# Autodesk Inventor assembly: fourbardraft
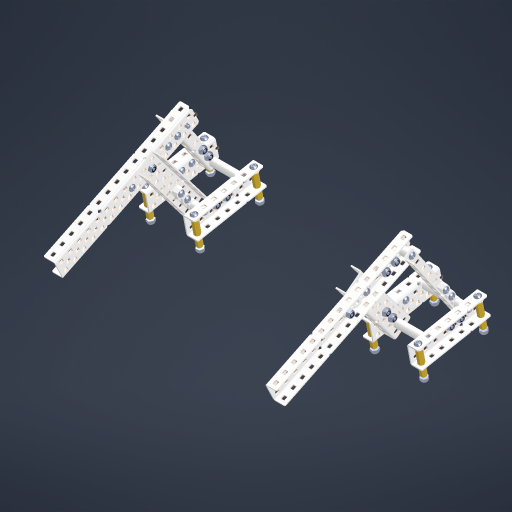
[picture p0: Inventor's stored thumbnail of the model, 512x512]
Saved by Autodesk Inventor 2023 (Build 270158000, 158)
## iProperties
Created: 2023-08-09
Part Number: fourbardraft
Document SubType Name: Assembly
Designer: srbel
Author: srbel
## Documents named in this file (28)
- C:\CAD\OverUnderCAD\Drive\fourbardraft.iam
- C:\CAD\OverUnderCAD\VEX-CAD-Inventor-1.4.0\Structure\C Channel\Aluminum 1x2x1\Alu C 1x2x1x6.ipt
- C:\CAD\OverUnderCAD\VEX-CAD-Inventor-1.4.0\Motion\Spacers\Spacer Nylon .313 OD\NSpacer .313 OD x .250.ipt
- C:\CAD\OverUnderCAD\VEX-CAD-Inventor-1.4.0\Motion\Spacers\Spacer Nylon .313 OD.ipt
- C:\CAD\OverUnderCAD\VEX-CAD-Inventor-1.4.0\Motion\Spacers\Spacer Nylon .313 OD\NSpacer .313 OD x .375.ipt
- C:\CAD\OverUnderCAD\VEX-CAD-Inventor-1.4.0\Motion\Spacers\Washer Teflon\TWasher .375 OD x .06250.ipt
- C:\CAD\OverUnderCAD\VEX-CAD-Inventor-1.4.0\Motion\Spacers\Washer Teflon.ipt
- C:\CAD\OverUnderCAD\VEX-CAD-Inventor-1.4.0\Structure\Hardware\Screw Steel - Star\SScrew Star Threaded .500.ipt
- C:\CAD\OverUnderCAD\VEX-CAD-Inventor-1.4.0\Structure\Hardware\Screw Steel - Star.ipt
- C:\CAD\OverUnderCAD\VEX-CAD-Inventor-1.4.0\Structure\Hardware\Screw Steel - Star\SScrew Star Threaded 2.500.ipt
- C:\CAD\OverUnderCAD\VEX-CAD-Inventor-1.4.0\Motion\Spacers\Spacer Nylon .313 OD\NSpacer .313 OD x .500.ipt
- C:\CAD\OverUnderCAD\VEX-CAD-Inventor-1.4.0\Structure\Hardware\Screw Steel - Star\SScrew Star Threaded .875.ipt
- C:\CAD\OverUnderCAD\Drive\fourbarintakebearing_MIR2.iam
- C:\CAD\OverUnderCAD\Drive\fourbarintakebearing_MIR_MIR1.iam
- C:\CAD\OverUnderCAD\VEX-CAD-Inventor-1.4.0\Motion\Shaft LS\Bearing Flat_MIR5.ipt
- C:\CAD\OverUnderCAD\VEX-CAD-Inventor-1.4.0\Structure\C Channel\Aluminum 1x2x1\Alu C 1x2x1x8_MIR2.ipt
- C:\CAD\OverUnderCAD\VEX-CAD-Inventor-1.4.0\Structure\Angle\Aluminum\1x1\Alu Angle 1x1x8_MIR2.ipt
- C:\CAD\OverUnderCAD\VEX-CAD-Inventor-1.4.0\Structure\C Channel\Aluminum 1x2x1\Alu C 1x2x1x15_MIR1.ipt
- C:\CAD\OverUnderCAD\VEX-CAD-Inventor-1.4.0\Motion\Shaft LS\Bearing Flat_MIR3_MIR1.ipt
- C:\CAD\OverUnderCAD\VEX-CAD-Inventor-1.4.0\Structure\Hardware\Nut Thin Nylock_MIR7_MIR1.ipt
- C:\CAD\OverUnderCAD\Drive\fourbarintakebearing_MIR2_MIR1.iam
- C:\CAD\OverUnderCAD\Drive\fourbarintakebearing_MIR_MIR1_MIR1.iam
- C:\CAD\OverUnderCAD\VEX-CAD-Inventor-1.4.0\Motion\Shaft LS\Bearing Flat_MIR5_MIR1.ipt
- C:\CAD\OverUnderCAD\VEX-CAD-Inventor-1.4.0\Structure\C Channel\Aluminum 1x2x1\Alu C 1x2x1x8_MIR2_MIR1.ipt
- C:\CAD\OverUnderCAD\VEX-CAD-Inventor-1.4.0\Structure\Angle\Aluminum\1x1\Alu Angle 1x1x8_MIR2_MIR1.ipt
- C:\CAD\OverUnderCAD\VEX-CAD-Inventor-1.4.0\Structure\C Channel\Aluminum 1x2x1\Alu C 1x2x1x15_MIR1_MIR1.ipt
- C:\CAD\OverUnderCAD\VEX-CAD-Inventor-1.4.0\Motion\Shaft LS\Bearing Flat_MIR3_MIR1_MIR1.ipt
- C:\CAD\OverUnderCAD\VEX-CAD-Inventor-1.4.0\Structure\Hardware\Nut Thin Nylock_MIR7_MIR1_MIR1.ipt
## Components (93 placed, 24 different names)
1. Alu C 1x2x1x6:1
2. fourbarintakebearing_MIR2:1 [sub-assembly] — Insert:64, Insert:91, Insert:94, Insert:164
3. fourbarintakebearing_MIR_MIR1:1 [sub-assembly] — Insert:68, Insert:76, Insert:78, Insert:79, Insert:90, Insert:168
4. Bearing Flat_MIR5:1 — Insert:62, Insert:63, Insert:65, Insert:85, Insert:86
5. Alu C 1x2x1x8_MIR2:1 — Insert:62, Insert:63, Insert:70, Insert:87, Insert:88, Insert:165, Insert:221, Insert:222
6. NSpacer .313 OD x .250:12 — Insert:64, Insert:65
7. Bearing Flat_MIR5:2 — Insert:66, Insert:67, Insert:69, Insert:82, Insert:83
8. Alu Angle 1x1x8_MIR2:1 — Insert:66, Insert:67, Insert:73, Insert:81, Insert:84, Insert:95, Insert:103
9. NSpacer .313 OD x .250:13 — Insert:68, Insert:69
10. Alu C 1x2x1x15_MIR1:1 — Insert:70, Insert:71, Insert:72, Insert:105, Insert:107, Insert:110, Insert:113, Insert:169
11. Bearing Flat_MIR5:3 — Insert:71, Insert:72, Insert:106, Insert:108, Insert:163
12. NSpacer .313 OD x .375:14 — Insert:73, Insert:163
13. Bearing Flat_MIR3_MIR1:1 — Insert:76, Insert:77, Insert:80, Insert:93
14. Nut Thin Nylock_MIR7_MIR1:1 — Insert:77
15. SScrew Star Threaded .500:15 — Insert:78
16. SScrew Star Threaded .500:16 — Insert:79
17. Nut Thin Nylock_MIR7_MIR1:2 — Insert:80
18. Nut Thin Nylock_MIR7_MIR1:3 — Insert:81
19. SScrew Star Threaded .500:17 — Insert:82
20. SScrew Star Threaded .500:18 — Insert:83
21. Nut Thin Nylock_MIR7_MIR1:4 — Insert:84
22. SScrew Star Threaded .500:19 — Insert:85
23. SScrew Star Threaded .500:20 — Insert:86
24. Nut Thin Nylock_MIR7_MIR1:5 — Insert:87
25. Nut Thin Nylock_MIR7_MIR1:6 — Insert:88
26. Nut Thin Nylock_MIR7_MIR1:7 — Insert:89
27. TWasher .375 OD x .06250:7 — Insert:89, Insert:90
28. Nut Thin Nylock_MIR7_MIR1:8 — Insert:92
29. TWasher .375 OD x .06250:8 — Insert:91, Insert:92
30. SScrew Star Threaded 2.500:21 — Insert:93
31. SScrew Star Threaded 2.500:22 — Insert:94
32. NSpacer .313 OD x .250:15 — Insert:96, Insert:164
33. NSpacer .313 OD x .500:16 — Insert:95, Insert:97
34. NSpacer .313 OD x .500:17 — Insert:96, Insert:97
35. SScrew Star Threaded .875:23 — Insert:103
36. SScrew Star Threaded .500:24 — Insert:105
37. Nut Thin Nylock_MIR7_MIR1:10 — Insert:106
38. SScrew Star Threaded .500:25 — Insert:107
39. Nut Thin Nylock_MIR7_MIR1:11 — Insert:108
40. SScrew Star Threaded .500:26 — Insert:109, Insert:112
41. Nut Thin Nylock_MIR7_MIR1:12 — Insert:109
42. SScrew Star Threaded .500:27 — Insert:110, Insert:111
43. Nut Thin Nylock_MIR7_MIR1:13 — Insert:111
44. Bearing Flat_MIR5:4 — Insert:112, Insert:113, Insert:169
45. NSpacer .313 OD x .500:30 — Insert:165, Insert:166
46. NSpacer .313 OD x .250:31 — Insert:166, Insert:167
47. NSpacer .313 OD x .500:32 — Insert:167, Insert:168
48. fourbarintakebearing_MIR2_MIR1:1 [sub-assembly] — Insert:173, Insert:199, Insert:201, Insert:202
49. fourbarintakebearing_MIR_MIR1_MIR1:1 [sub-assembly] — Insert:177, Insert:183, Insert:185, Insert:186, Insert:196, Insert:219
50. Bearing Flat_MIR5_MIR1:1 — Insert:170, Insert:171, Insert:172, Insert:192, Insert:193
51. Alu C 1x2x1x8_MIR2_MIR1:1 — Insert:170, Insert:171, Insert:178, Insert:194, Insert:195, Insert:217, Insert:221, Insert:222
52. NSpacer .313 OD x .250:33 — Insert:172, Insert:173
53. Bearing Flat_MIR5_MIR1:2 — Insert:174, Insert:175, Insert:176, Insert:189, Insert:190
54. Alu Angle 1x1x8_MIR2_MIR1:1 — Insert:174, Insert:175, Insert:182, Insert:188, Insert:191, Insert:203, Insert:206
55. NSpacer .313 OD x .250:34 — Insert:176, Insert:177
56. Alu C 1x2x1x15_MIR1_MIR1:1 — Insert:178, Insert:179, Insert:180, Insert:207, Insert:209, Insert:212, Insert:214, Insert:215
57. Bearing Flat_MIR5_MIR1:3 — Insert:179, Insert:180, Insert:181, Insert:208, Insert:210
58. NSpacer .313 OD x .375:35 — Insert:181, Insert:182
59. Bearing Flat_MIR3_MIR1_MIR1:1 — Insert:183, Insert:184, Insert:187, Insert:200
60. Nut Thin Nylock_MIR7_MIR1_MIR1:1 — Insert:184
61. SScrew Star Threaded .500:28 — Insert:185
62. SScrew Star Threaded .500:29 — Insert:186
63. Nut Thin Nylock_MIR7_MIR1_MIR1:2 — Insert:187
64. Nut Thin Nylock_MIR7_MIR1_MIR1:3 — Insert:188
65. SScrew Star Threaded .500:30 — Insert:189
66. SScrew Star Threaded .500:31 — Insert:190
67. Nut Thin Nylock_MIR7_MIR1_MIR1:4 — Insert:191
68. SScrew Star Threaded .500:32 — Insert:192
69. SScrew Star Threaded .500:33 — Insert:193
70. Nut Thin Nylock_MIR7_MIR1_MIR1:5 — Insert:194
71. Nut Thin Nylock_MIR7_MIR1_MIR1:6 — Insert:195
72. Nut Thin Nylock_MIR7_MIR1_MIR1:7 — Insert:197
73. TWasher .375 OD x .06250:9 — Insert:196, Insert:197
74. Nut Thin Nylock_MIR7_MIR1_MIR1:8 — Insert:198
75. TWasher .375 OD x .06250:10 — Insert:198, Insert:199
76. SScrew Star Threaded 2.500:34 — Insert:200
77. SScrew Star Threaded 2.500:35 — Insert:201
78. NSpacer .313 OD x .250:36 — Insert:202, Insert:205
79. NSpacer .313 OD x .500:37 — Insert:203, Insert:204
80. NSpacer .313 OD x .500:38 — Insert:204, Insert:205
81. SScrew Star Threaded .875:36 — Insert:206
82. SScrew Star Threaded .500:37 — Insert:207
83. Nut Thin Nylock_MIR7_MIR1_MIR1:9 — Insert:208
84. SScrew Star Threaded .500:38 — Insert:209
85. Nut Thin Nylock_MIR7_MIR1_MIR1:10 — Insert:210
86. SScrew Star Threaded .500:39 — Insert:211, Insert:216
87. Nut Thin Nylock_MIR7_MIR1_MIR1:11 — Insert:211
88. SScrew Star Threaded .500:40 — Insert:212, Insert:213
89. Nut Thin Nylock_MIR7_MIR1_MIR1:12 — Insert:213
90. Bearing Flat_MIR5_MIR1:4 — Insert:214, Insert:215, Insert:216
91. NSpacer .313 OD x .500:39 — Insert:217, Insert:218
92. NSpacer .313 OD x .250:40 — Insert:218, Insert:220
93. NSpacer .313 OD x .500:41 — Insert:219, Insert:220
## Relationships (104: Insert 104)
- Insert:62: Bearing Flat_MIR5:1 ↔ Alu C 1x2x1x8_MIR2:1
- Insert:63: Bearing Flat_MIR5:1 ↔ Alu C 1x2x1x8_MIR2:1
- Insert:64: fourbarintakebearing_MIR2:1 ↔ NSpacer .313 OD x .250:12
- Insert:65: Bearing Flat_MIR5:1 ↔ NSpacer .313 OD x .250:12
- Insert:66: Bearing Flat_MIR5:2 ↔ Alu Angle 1x1x8_MIR2:1
- Insert:67: Bearing Flat_MIR5:2 ↔ Alu Angle 1x1x8_MIR2:1
- Insert:68: fourbarintakebearing_MIR_MIR1:1 ↔ NSpacer .313 OD x .250:13
- Insert:69: Bearing Flat_MIR5:2 ↔ NSpacer .313 OD x .250:13
- Insert:70: Alu C 1x2x1x8_MIR2:1 ↔ Alu C 1x2x1x15_MIR1:1
- Insert:71: Alu C 1x2x1x15_MIR1:1 ↔ Bearing Flat_MIR5:3
- Insert:72: Alu C 1x2x1x15_MIR1:1 ↔ Bearing Flat_MIR5:3
- Insert:73: Alu Angle 1x1x8_MIR2:1 ↔ NSpacer .313 OD x .375:14
- Insert:76: fourbarintakebearing_MIR_MIR1:1 ↔ Bearing Flat_MIR3_MIR1:1
- Insert:77: Bearing Flat_MIR3_MIR1:1 ↔ Nut Thin Nylock_MIR7_MIR1:1
- Insert:78: fourbarintakebearing_MIR_MIR1:1 ↔ SScrew Star Threaded .500:15
- Insert:79: fourbarintakebearing_MIR_MIR1:1 ↔ SScrew Star Threaded .500:16
- Insert:80: Bearing Flat_MIR3_MIR1:1 ↔ Nut Thin Nylock_MIR7_MIR1:2
- Insert:81: Alu Angle 1x1x8_MIR2:1 ↔ Nut Thin Nylock_MIR7_MIR1:3
- Insert:82: Bearing Flat_MIR5:2 ↔ SScrew Star Threaded .500:17
- Insert:83: Bearing Flat_MIR5:2 ↔ SScrew Star Threaded .500:18
- Insert:84: Alu Angle 1x1x8_MIR2:1 ↔ Nut Thin Nylock_MIR7_MIR1:4
- Insert:85: Bearing Flat_MIR5:1 ↔ SScrew Star Threaded .500:19
- Insert:86: Bearing Flat_MIR5:1 ↔ SScrew Star Threaded .500:20
- Insert:87: Alu C 1x2x1x8_MIR2:1 ↔ Nut Thin Nylock_MIR7_MIR1:5
- Insert:88: Alu C 1x2x1x8_MIR2:1 ↔ Nut Thin Nylock_MIR7_MIR1:6
- Insert:89: Nut Thin Nylock_MIR7_MIR1:7 ↔ TWasher .375 OD x .06250:7
- Insert:90: fourbarintakebearing_MIR_MIR1:1 ↔ TWasher .375 OD x .06250:7
- Insert:91: fourbarintakebearing_MIR2:1 ↔ TWasher .375 OD x .06250:8
- Insert:92: Nut Thin Nylock_MIR7_MIR1:8 ↔ TWasher .375 OD x .06250:8
- Insert:93: Bearing Flat_MIR3_MIR1:1 ↔ SScrew Star Threaded 2.500:21
- Insert:94: fourbarintakebearing_MIR2:1 ↔ SScrew Star Threaded 2.500:22
- Insert:95: Alu Angle 1x1x8_MIR2:1 ↔ NSpacer .313 OD x .500:16
- Insert:96: NSpacer .313 OD x .250:15 ↔ NSpacer .313 OD x .500:17
- Insert:97: NSpacer .313 OD x .500:16 ↔ NSpacer .313 OD x .500:17
- Insert:103: Alu Angle 1x1x8_MIR2:1 ↔ SScrew Star Threaded .875:23
- Insert:105: Alu C 1x2x1x15_MIR1:1 ↔ SScrew Star Threaded .500:24
- Insert:106: Bearing Flat_MIR5:3 ↔ Nut Thin Nylock_MIR7_MIR1:10
- Insert:107: Alu C 1x2x1x15_MIR1:1 ↔ SScrew Star Threaded .500:25
- Insert:108: Bearing Flat_MIR5:3 ↔ Nut Thin Nylock_MIR7_MIR1:11
- Insert:109 (8.3185 mm): SScrew Star Threaded .500:26 ↔ Nut Thin Nylock_MIR7_MIR1:12
- Insert:110: Alu C 1x2x1x15_MIR1:1 ↔ SScrew Star Threaded .500:27
- Insert:111 (8.3185 mm): SScrew Star Threaded .500:27 ↔ Nut Thin Nylock_MIR7_MIR1:13
- Insert:112: SScrew Star Threaded .500:26 ↔ Bearing Flat_MIR5:4
- Insert:113: Alu C 1x2x1x15_MIR1:1 ↔ Bearing Flat_MIR5:4
- Insert:163: Bearing Flat_MIR5:3 ↔ NSpacer .313 OD x .375:14
- Insert:164: fourbarintakebearing_MIR2:1 ↔ NSpacer .313 OD x .250:15
- Insert:165: Alu C 1x2x1x8_MIR2:1 ↔ NSpacer .313 OD x .500:30
- Insert:166: NSpacer .313 OD x .500:30 ↔ NSpacer .313 OD x .250:31
- Insert:167: NSpacer .313 OD x .250:31 ↔ NSpacer .313 OD x .500:32
- Insert:168: fourbarintakebearing_MIR_MIR1:1 ↔ NSpacer .313 OD x .500:32
- Insert:169: Alu C 1x2x1x15_MIR1:1 ↔ Bearing Flat_MIR5:4
- Insert:170: Bearing Flat_MIR5_MIR1:1 ↔ Alu C 1x2x1x8_MIR2_MIR1:1
- Insert:171: Bearing Flat_MIR5_MIR1:1 ↔ Alu C 1x2x1x8_MIR2_MIR1:1
- Insert:172: Bearing Flat_MIR5_MIR1:1 ↔ NSpacer .313 OD x .250:33
- Insert:173: fourbarintakebearing_MIR2_MIR1:1 ↔ NSpacer .313 OD x .250:33
- Insert:174: Bearing Flat_MIR5_MIR1:2 ↔ Alu Angle 1x1x8_MIR2_MIR1:1
- Insert:175: Bearing Flat_MIR5_MIR1:2 ↔ Alu Angle 1x1x8_MIR2_MIR1:1
- Insert:176: Bearing Flat_MIR5_MIR1:2 ↔ NSpacer .313 OD x .250:34
- Insert:177: fourbarintakebearing_MIR_MIR1_MIR1:1 ↔ NSpacer .313 OD x .250:34
- Insert:178: Alu C 1x2x1x8_MIR2_MIR1:1 ↔ Alu C 1x2x1x15_MIR1_MIR1:1
- Insert:179: Alu C 1x2x1x15_MIR1_MIR1:1 ↔ Bearing Flat_MIR5_MIR1:3
- Insert:180: Alu C 1x2x1x15_MIR1_MIR1:1 ↔ Bearing Flat_MIR5_MIR1:3
- Insert:181: Bearing Flat_MIR5_MIR1:3 ↔ NSpacer .313 OD x .375:35
- Insert:182: Alu Angle 1x1x8_MIR2_MIR1:1 ↔ NSpacer .313 OD x .375:35
- Insert:183: fourbarintakebearing_MIR_MIR1_MIR1:1 ↔ Bearing Flat_MIR3_MIR1_MIR1:1
- Insert:184: Bearing Flat_MIR3_MIR1_MIR1:1 ↔ Nut Thin Nylock_MIR7_MIR1_MIR1:1
- Insert:185: fourbarintakebearing_MIR_MIR1_MIR1:1 ↔ SScrew Star Threaded .500:28
- Insert:186: fourbarintakebearing_MIR_MIR1_MIR1:1 ↔ SScrew Star Threaded .500:29
- Insert:187: Bearing Flat_MIR3_MIR1_MIR1:1 ↔ Nut Thin Nylock_MIR7_MIR1_MIR1:2
- Insert:188: Alu Angle 1x1x8_MIR2_MIR1:1 ↔ Nut Thin Nylock_MIR7_MIR1_MIR1:3
- Insert:189: Bearing Flat_MIR5_MIR1:2 ↔ SScrew Star Threaded .500:30
- Insert:190: Bearing Flat_MIR5_MIR1:2 ↔ SScrew Star Threaded .500:31
- Insert:191: Alu Angle 1x1x8_MIR2_MIR1:1 ↔ Nut Thin Nylock_MIR7_MIR1_MIR1:4
- Insert:192: Bearing Flat_MIR5_MIR1:1 ↔ SScrew Star Threaded .500:32
- Insert:193: Bearing Flat_MIR5_MIR1:1 ↔ SScrew Star Threaded .500:33
- Insert:194: Alu C 1x2x1x8_MIR2_MIR1:1 ↔ Nut Thin Nylock_MIR7_MIR1_MIR1:5
- Insert:195: Alu C 1x2x1x8_MIR2_MIR1:1 ↔ Nut Thin Nylock_MIR7_MIR1_MIR1:6
- Insert:196: fourbarintakebearing_MIR_MIR1_MIR1:1 ↔ TWasher .375 OD x .06250:9
- Insert:197: Nut Thin Nylock_MIR7_MIR1_MIR1:7 ↔ TWasher .375 OD x .06250:9
- Insert:198: Nut Thin Nylock_MIR7_MIR1_MIR1:8 ↔ TWasher .375 OD x .06250:10
- Insert:199: fourbarintakebearing_MIR2_MIR1:1 ↔ TWasher .375 OD x .06250:10
- Insert:200: Bearing Flat_MIR3_MIR1_MIR1:1 ↔ SScrew Star Threaded 2.500:34
- Insert:201: fourbarintakebearing_MIR2_MIR1:1 ↔ SScrew Star Threaded 2.500:35
- Insert:202: fourbarintakebearing_MIR2_MIR1:1 ↔ NSpacer .313 OD x .250:36
- Insert:203: Alu Angle 1x1x8_MIR2_MIR1:1 ↔ NSpacer .313 OD x .500:37
- Insert:204: NSpacer .313 OD x .500:37 ↔ NSpacer .313 OD x .500:38
- Insert:205: NSpacer .313 OD x .250:36 ↔ NSpacer .313 OD x .500:38
- Insert:206: Alu Angle 1x1x8_MIR2_MIR1:1 ↔ SScrew Star Threaded .875:36
- Insert:207: Alu C 1x2x1x15_MIR1_MIR1:1 ↔ SScrew Star Threaded .500:37
- Insert:208: Bearing Flat_MIR5_MIR1:3 ↔ Nut Thin Nylock_MIR7_MIR1_MIR1:9
- Insert:209: Alu C 1x2x1x15_MIR1_MIR1:1 ↔ SScrew Star Threaded .500:38
- Insert:210: Bearing Flat_MIR5_MIR1:3 ↔ Nut Thin Nylock_MIR7_MIR1_MIR1:10
- Insert:211 (8.3185 mm): SScrew Star Threaded .500:39 ↔ Nut Thin Nylock_MIR7_MIR1_MIR1:11
- Insert:212: Alu C 1x2x1x15_MIR1_MIR1:1 ↔ SScrew Star Threaded .500:40
- Insert:213 (8.3185 mm): SScrew Star Threaded .500:40 ↔ Nut Thin Nylock_MIR7_MIR1_MIR1:12
- Insert:214: Alu C 1x2x1x15_MIR1_MIR1:1 ↔ Bearing Flat_MIR5_MIR1:4
- Insert:215: Alu C 1x2x1x15_MIR1_MIR1:1 ↔ Bearing Flat_MIR5_MIR1:4
- Insert:216: SScrew Star Threaded .500:39 ↔ Bearing Flat_MIR5_MIR1:4
- Insert:217: Alu C 1x2x1x8_MIR2_MIR1:1 ↔ NSpacer .313 OD x .500:39
- Insert:218: NSpacer .313 OD x .500:39 ↔ NSpacer .313 OD x .250:40
- Insert:219: fourbarintakebearing_MIR_MIR1_MIR1:1 ↔ NSpacer .313 OD x .500:41
- Insert:220: NSpacer .313 OD x .250:40 ↔ NSpacer .313 OD x .500:41
- Insert:221 (260.3496 mm): Alu C 1x2x1x8_MIR2:1 ↔ Alu C 1x2x1x8_MIR2_MIR1:1
- Insert:222 (260.3496 mm): Alu C 1x2x1x8_MIR2:1 ↔ Alu C 1x2x1x8_MIR2_MIR1:1
